# Autodesk Inventor assembly: frame
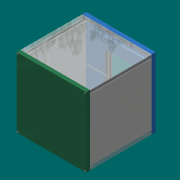
[picture p0: Inventor's stored thumbnail of the model, 180x180]
Saved by Autodesk Inventor 2016 (Build 200138000, 138)
## iProperties
Created: 2015-10-13
Part Number: frame
Document SubType Name: Assembly
Designer: Sawaiz
Author: Sawaiz
## Documents named in this file (7)
- C:\Users\Sawaiz\OneDrive\projects\modularRICH\frame\frame.iam
- C:\Users\Sawaiz\OneDrive\projects\modularRICH\frame\sides.ipt
- C:\Users\Sawaiz\OneDrive\projects\modularRICH\frame\back.iam
- C:\Users\Sawaiz\OneDrive\projects\modularRICH\frame\front.iam
- C:\Users\Sawaiz\OneDrive\projects\modularRICH\frame\topBottom.iam
- C:\Users\Sawaiz\OneDrive\projects\modularRICH\frame\0x0.625flatPhilips.ipt
- C:\Users\Sawaiz\OneDrive\projects\modularRICH\modularRICH.xlsx
## Components (14 placed, 5 different names)
1. back:1 [sub-assembly] — Flush:1, Flush:2, Mate:1, Mate:7, Mate:8, Flush:9, Mate:9, Mate:10, Mate:11, Mate:12, Mate:13, Mate:14, Mate:15, Flush:10, Flush:11, Flush:12, Flush:13, Flush:14, Flush:15, Flush:16
2. front:1 [sub-assembly] — Flush:1, Flush:2, Flush:3, Flush:4, Flush:6, Mate:2, Mate:3, Mate:17
3. topBottom:1 [sub-assembly] — Flush:4, Flush:5, Flush:6, Mate:1, Mate:3
4. topBottom:2 [sub-assembly] — Flush:3, Flush:5, Mate:2, Flush:7, Mate:6, Flush:8, Mate:16
5. sides:1 — Mate:6, Mate:7, Flush:8
6. sides:2 — Flush:7, Mate:16, Mate:17
7. 0x0.625flatPhilips:1 — Mate:8, Flush:9
8. 0x0.625flatPhilips:2 — Mate:9, Flush:15
9. 0x0.625flatPhilips:3 — Mate:10, Flush:16
10. 0x0.625flatPhilips:4 — Mate:11, Flush:14
11. 0x0.625flatPhilips:5 — Mate:15, Flush:10
12. 0x0.625flatPhilips:6 — Mate:14, Flush:11
13. 0x0.625flatPhilips:7 — Mate:12, Flush:13
14. 0x0.625flatPhilips:8 — Mate:13, Flush:12
## Relationships (31: Flush 16, Mate 15)
- Flush:1: back:1 ↔ front:1
- Flush:2: back:1 ↔ front:1
- Flush:3: front:1 ↔ topBottom:2
- Flush:4: front:1 ↔ topBottom:1
- Flush:5: topBottom:1 ↔ topBottom:2
- Flush:6: front:1 ↔ topBottom:1
- Mate:1: back:1 ↔ topBottom:1
- Mate:2: front:1 ↔ topBottom:2
- Mate:3: front:1 ↔ topBottom:1
- Flush:7: topBottom:2 ↔ sides:2
- Mate:6: topBottom:2 ↔ sides:1
- Mate:7: back:1 ↔ sides:1
- Flush:8: topBottom:2 ↔ sides:1
- Mate:8: back:1 ↔ 0x0.625flatPhilips:1
- Flush:9: back:1 ↔ 0x0.625flatPhilips:1
- Mate:9: back:1 ↔ 0x0.625flatPhilips:2
- Mate:10: back:1 ↔ 0x0.625flatPhilips:3
- Mate:11: back:1 ↔ 0x0.625flatPhilips:4
- Mate:12: back:1 ↔ 0x0.625flatPhilips:7
- Mate:13: back:1 ↔ 0x0.625flatPhilips:8
- Mate:14: back:1 ↔ 0x0.625flatPhilips:6
- Mate:15: back:1 ↔ 0x0.625flatPhilips:5
- Flush:10: back:1 ↔ 0x0.625flatPhilips:5
- Flush:11: back:1 ↔ 0x0.625flatPhilips:6
- Flush:12: back:1 ↔ 0x0.625flatPhilips:8
- Flush:13: back:1 ↔ 0x0.625flatPhilips:7
- Flush:14: back:1 ↔ 0x0.625flatPhilips:4
- Flush:15: back:1 ↔ 0x0.625flatPhilips:2
- Flush:16: back:1 ↔ 0x0.625flatPhilips:3
- Mate:16: topBottom:2 ↔ sides:2
- Mate:17: front:1 ↔ sides:2
## Named parameters: acrylicThickness = 6.35 mm, aerogelThickness = 20 mm, height = 101.6 mm, width = 101.6 mm, depth = 101.6 mm, mirrorAngle = 5 deg, detectorWidth = 52 mm, detectorHeight = 52 mm, mirrorThickness = 3 mm, fresnelThickness = 0.1 mm, grooveDensity = 100, focalLength = 76.2 mm, ior = 1.49, centerThickness = 1.524 mm, fresnelAngle = 90 deg, fresnelEffectiveDiameter = 76.2 mm, mirrorSuppourtWidth = 38.1 mm, backGrooveBit = 4.8006 mm, sensorHolderWidth = 88.9 mm, sensorHolderSensorWidth = 53.975 mm, sensorHolderSesnorHeight = 53.975 mm, sensorHolderHeight = 88.9 mm, sensorHolderSensorHeight = 53.975 mm, sensorHolderORingGroove = 3.175 mm, sensorHolderORing = 3.175 mm, sensorHolderFlushORingID = 254 mm, sensorHolderFlushORing = 3.175 mm, frontBackORingID = 419.1 mm, oRingWidth = 3.175 mm, sensorHolderORingID = 203.2 mm, topBottomHorizontalMirrorGroove = 12.7 mm, backMirrorGroove = 6.35 mm, mirrorGroove = 19.05 mm, compressionPercent = 40, fresnelChamfer = 6.35 mm, mirrorGrooveFillet = 6.35 mm, mirrorGrooveDrill = 6.35 mm, mirrorGrooveMill = 3.175 mm
